# Autodesk Inventor assembly: MK3 Billet Wheel Assembly
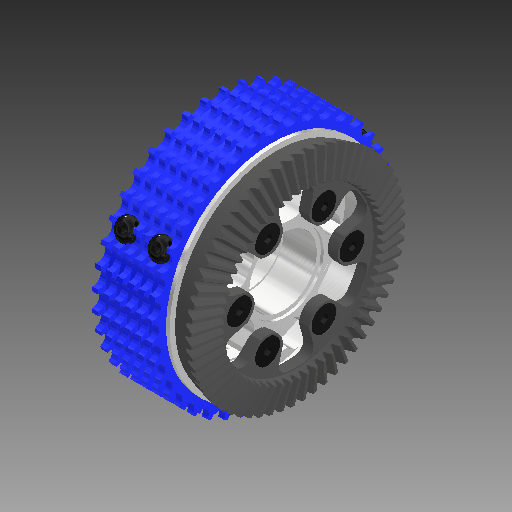
[picture p0: Inventor's stored thumbnail of the model, 512x512]
Saved by Autodesk Inventor 2025 (Build 290162010, 162A)
## iProperties
Created: 2024-07-20
Part Number: MK3 Billet Wheel Assembly
Document SubType Name: Assembly
Designer: rohan
Author: rohan
## Documents named in this file (7)
- D:\ultimate-hecker\Computer-Aided-Design\FRC-Offseason-Design-Training\Parts Library\Drivetrains\Swerve Modules\MK3\MK3 Billet Wheel Assembly.iam
- D:\ultimate-hecker\Computer-Aided-Design\FRC-Offseason-Design-Training\Parts Library\Wheels\Billet Wheels\Billet Wheel 4in X 1in.ipt
- D:\ultimate-hecker\Computer-Aided-Design\FRC-Offseason-Design-Training\Parts Library\Wheels\Billet Wheels\Blue Nitrile Thread 4in X 1in.ipt
- D:\ultimate-hecker\Computer-Aided-Design\FRC-Offseason-Design-Training\Parts Library\Hardware\Fasteners\Machine Screws.ipt
- D:\ultimate-hecker\Computer-Aided-Design\FRC-Offseason-Design-Training\Parts Library\Hardware\Fasteners\Machine Screws\10-32 UNFx0.5 Button Head Cap Screw.ipt
- D:\ultimate-hecker\Computer-Aided-Design\FRC-Offseason-Design-Training\Parts Library\Power Transfer\Gears (Bevel)\Bevel Gear KSB1.5-6015 (VersaHub).ipt
- D:\ultimate-hecker\Computer-Aided-Design\FRC-Offseason-Design-Training\Parts Library\Hardware\Fasteners\Machine Screws\10-32 UNFx0.5 Countersunk Machine Screw.ipt
## Components (17 placed, 5 different names)
1. Billet Wheel 4in X 1in:1 — Mate:1, Mate:2, Insert:9, Insert:10
2. Blue Nitrile Thread 4in X 1in:1 — Mate:1, Mate:2, Insert:1, Insert:2, Insert:3, Insert:4, Insert:5, Insert:6, Insert:7, Insert:8
3. 10-32 UNFx0.5 Button Head Cap Screw:2 — Insert:3
4. 10-32 UNFx0.5 Button Head Cap Screw:3 — Insert:4
5. 10-32 UNFx0.5 Button Head Cap Screw:4 — Insert:7
6. 10-32 UNFx0.5 Button Head Cap Screw:5 — Insert:5
7. 10-32 UNFx0.5 Button Head Cap Screw:6 — Insert:1
8. 10-32 UNFx0.5 Button Head Cap Screw:7 — Insert:2
9. 10-32 UNFx0.5 Button Head Cap Screw:8 — Insert:6
10. 10-32 UNFx0.5 Button Head Cap Screw:9 — Insert:8
11. Bevel Gear KSB1.5-6015 (VersaHub):1 — Insert:9, Insert:10, Flush:1, Mate:3, Flush:2, Flush:3, Flush:4, Flush:5, Flush:6, Mate:4, Mate:5, Mate:6, Mate:7, Mate:8
12. 10-32 UNFx0.5 Countersunk Machine Screw:10 — Flush:5, Mate:6
13. 10-32 UNFx0.5 Countersunk Machine Screw:11 — Flush:3, Mate:7
14. 10-32 UNFx0.5 Countersunk Machine Screw:12 — Flush:2, Mate:8
15. 10-32 UNFx0.5 Countersunk Machine Screw:13 — Flush:1, Mate:3
16. 10-32 UNFx0.5 Countersunk Machine Screw:14 — Flush:4, Mate:5
17. 10-32 UNFx0.5 Countersunk Machine Screw:15 — Flush:6, Mate:4
## Relationships (24: Insert 10, Mate 8, Flush 6)
- Mate:1: Billet Wheel 4in X 1in:1 ↔ Blue Nitrile Thread 4in X 1in:1
- Mate:2: Billet Wheel 4in X 1in:1 ↔ Blue Nitrile Thread 4in X 1in:1
- Insert:1: Blue Nitrile Thread 4in X 1in:1 ↔ 10-32 UNFx0.5 Button Head Cap Screw:6
- Insert:2: Blue Nitrile Thread 4in X 1in:1 ↔ 10-32 UNFx0.5 Button Head Cap Screw:7
- Insert:3: Blue Nitrile Thread 4in X 1in:1 ↔ 10-32 UNFx0.5 Button Head Cap Screw:2
- Insert:4: Blue Nitrile Thread 4in X 1in:1 ↔ 10-32 UNFx0.5 Button Head Cap Screw:3
- Insert:5: Blue Nitrile Thread 4in X 1in:1 ↔ 10-32 UNFx0.5 Button Head Cap Screw:5
- Insert:6: Blue Nitrile Thread 4in X 1in:1 ↔ 10-32 UNFx0.5 Button Head Cap Screw:8
- Insert:7: Blue Nitrile Thread 4in X 1in:1 ↔ 10-32 UNFx0.5 Button Head Cap Screw:4
- Insert:8: Blue Nitrile Thread 4in X 1in:1 ↔ 10-32 UNFx0.5 Button Head Cap Screw:9
- Insert:9: Billet Wheel 4in X 1in:1 ↔ Bevel Gear KSB1.5-6015 (VersaHub):1
- Insert:10: Billet Wheel 4in X 1in:1 ↔ Bevel Gear KSB1.5-6015 (VersaHub):1
- Flush:1 (0.127 mm): Bevel Gear KSB1.5-6015 (VersaHub):1 ↔ 10-32 UNFx0.5 Countersunk Machine Screw:13
- Mate:3: Bevel Gear KSB1.5-6015 (VersaHub):1 ↔ 10-32 UNFx0.5 Countersunk Machine Screw:13
- Flush:2 (0.127 mm): Bevel Gear KSB1.5-6015 (VersaHub):1 ↔ 10-32 UNFx0.5 Countersunk Machine Screw:12
- Flush:3 (0.127 mm): Bevel Gear KSB1.5-6015 (VersaHub):1 ↔ 10-32 UNFx0.5 Countersunk Machine Screw:11
- Flush:4 (0.127 mm): Bevel Gear KSB1.5-6015 (VersaHub):1 ↔ 10-32 UNFx0.5 Countersunk Machine Screw:14
- Flush:5 (0.127 mm): Bevel Gear KSB1.5-6015 (VersaHub):1 ↔ 10-32 UNFx0.5 Countersunk Machine Screw:10
- Flush:6 (0.127 mm): Bevel Gear KSB1.5-6015 (VersaHub):1 ↔ 10-32 UNFx0.5 Countersunk Machine Screw:15
- Mate:4: Bevel Gear KSB1.5-6015 (VersaHub):1 ↔ 10-32 UNFx0.5 Countersunk Machine Screw:15
- Mate:5: Bevel Gear KSB1.5-6015 (VersaHub):1 ↔ 10-32 UNFx0.5 Countersunk Machine Screw:14
- Mate:6: Bevel Gear KSB1.5-6015 (VersaHub):1 ↔ 10-32 UNFx0.5 Countersunk Machine Screw:10
- Mate:7: Bevel Gear KSB1.5-6015 (VersaHub):1 ↔ 10-32 UNFx0.5 Countersunk Machine Screw:11
- Mate:8: Bevel Gear KSB1.5-6015 (VersaHub):1 ↔ 10-32 UNFx0.5 Countersunk Machine Screw:12
